# Autodesk Inventor assembly: SirHexAlot
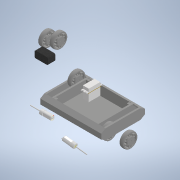
[picture p0: Inventor's stored thumbnail of the model, 180x180]
Saved by Autodesk Inventor 2020 (Build 240168000, 168)
## iProperties
Created: 2023-12-21
Part Number: SirHexAlot
Document SubType Name: Assembly
Designer: smz3rm
Mass: 469.52 g
Surface Area: 1790.41 cm^2
Volume: 428.698 cm^3
Density: 1.09522 g/cm^3
Author: smz3rm
## Documents named in this file (9)
- C:\Users\smz3rm\OneDrive - BP\Documents\DigitalTwin\Models\BattleBot\Flipper\SirHexAlot.iam
- C:\Users\smz3rm\OneDrive - BP\Documents\DigitalTwin\Models\BattleBot\Flipper\HexBody.ipt
- C:\Users\smz3rm\OneDrive - BP\Documents\DigitalTwin\Models\BattleBot\Flipper\HexWheelGuard.ipt
- C:\Users\smz3rm\OneDrive - BP\Documents\DigitalTwin\Models\BattleBot\Flipper\PulleyedWheelV1.ipt
- C:\Users\smz3rm\OneDrive - BP\Documents\DigitalTwin\Models\BattleBot\DriveMotorV2.ipt
- C:\Users\smz3rm\OneDrive - BP\Documents\DigitalTwin\Models\BattleBot\SwitchHolder.ipt
- C:\Users\smz3rm\OneDrive - BP\Documents\DigitalTwin\Models\BattleBot\Switch.ipt
- C:\Users\smz3rm\OneDrive - BP\Documents\DigitalTwin\Models\BattleBot\BatteryV1.ipt
- C:\Users\smz3rm\OneDrive - BP\Documents\DigitalTwin\Models\BattleBot\Flipper\Servo.ipt
## Components (14 placed, 8 different names)
1. HexBody:1 — Flush:1, Flush:2, Mate:1, Flush:3, Flush:4, Mate:2
2. HexWheelGuard:1 — Flush:1, Mate:1, Flush:3
3. PulleyedWheelV1:1
4. PulleyedWheelV1:2
5. PulleyedWheelV1:3
6. DriveMotorV2:1
7. DriveMotorV2:2
8. SwitchHolder:1
9. Switch:1
10. BatteryV1:1
11. PulleyedWheelV1:4
12. PulleyedWheelV1:5
13. HexWheelGuard:2 — Flush:2, Flush:4, Mate:2
14. Servo:1
## Relationships (6: Flush 4, Mate 2)
- Flush:1: HexBody:1 ↔ HexWheelGuard:1
- Flush:2: HexBody:1 ↔ HexWheelGuard:2
- Mate:1: HexBody:1 ↔ HexWheelGuard:1
- Flush:3: HexBody:1 ↔ HexWheelGuard:1
- Flush:4: HexBody:1 ↔ HexWheelGuard:2
- Mate:2: HexBody:1 ↔ HexWheelGuard:2
